# Autodesk Inventor assembly: Full_Auto_Robot_Assembly_V1.1_16.10.25
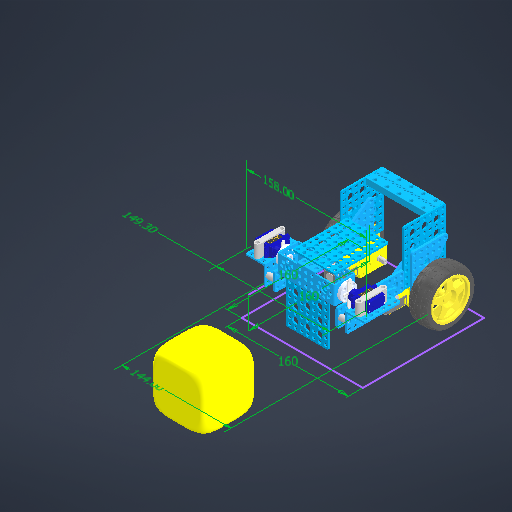
[picture p0: Inventor's stored thumbnail of the model, 512x512]
Saved by Autodesk Inventor 2026.1 (Build 301233020, 233B)
## iProperties
Created: 2025-10-11
Part Number: Full_Auto_Robot_Assembly_V1.1_16.10.25
Document SubType Name: Assembly
Designer: Asus
Author: Asus
## Documents named in this file (13)
- D:\KMITL\Computer_Programming\ComPro_Project\Robot_design_CAD_files\Full_Auto_Robot_Assembly_V1.1_16.10.25.iam
- D:\KMITL\Computer_Programming\ComPro_Project\Material_Parts_CAD_files\Metal_parts\Plate0324-088 V1.0.ipt
- D:\KMITL\Computer_Programming\ComPro_Project\Material_Parts_CAD_files\Metal_parts\Triangle Plate 6x8.ipt
- D:\KMITL\Computer_Programming\ComPro_Project\Material_Parts_CAD_files\Metal_parts\Beam0824-5.ipt
- D:\KMITL\Computer_Programming\ComPro_Project\Material_Parts_CAD_files\Metal_parts\Plate 7x9.ipt
- D:\KMITL\Computer_Programming\ComPro_Project\Material_Parts_CAD_files\Electronic_parts\yellow_dc_motor.ipt
- D:\KMITL\Computer_Programming\ComPro_Project\Material_Parts_CAD_files\Arudino_parts\Wheel D65x25.ipt
- D:\KMITL\Computer_Programming\ComPro_Project\Robot_design_CAD_files\Auto_robot_gate_mechanism_V1_11.10.25.iam
- D:\KMITL\Computer_Programming\ComPro_Project\Material_Parts_CAD_files\Metal_parts\Bracket 3x6.ipt
- D:\KMITL\Computer_Programming\ComPro_Project\Material_Parts_CAD_files\MakeX_parts\Standoff_010.ipt
- D:\KMITL\Computer_Programming\ComPro_Project\Field_materials_CAD_files\Objective_Block_Auto.ipt
- D:\KMITL\Computer_Programming\ComPro_Project\3D_Printing_Parts_CAD_files\Micro_servo_frame_2.ipt
- D:\KMITL\Computer_Programming\ComPro_Project\3D_Printing_Parts_CAD_files\Micro_servo_frame_1.ipt
## Components (25 placed, 12 different names)
1. Plate0324-088 V1.0:1 — Rigid:4, Mate:1, Mate:2, Mate:3, Mate:15, Tangent:1, Mate:18, Rigid:8, Rigid:9
2. Triangle Plate 6x8:1 — Rigid:4, Mate:1, Mate:2, Mate:3, Mate:4, Rigid:1
3. Beam0824-5:1 — Mate:6, Mate:7, Mate:8, Mate:11, Mate:12, Mate:13
4. Plate 7x9:1 — Mate:4, Rigid:1, Mate:5, Rigid:5, Mate:6, Mate:7, Mate:8
5. Triangle Plate 6x8:2 — Mate:5, Rigid:5, Mate:16
6. Plate0324-088 V1.0:2 — Rigid:6, Rigid:11, Rigid:12
7. Triangle Plate 6x8:3 — Rigid:6, Rotational:1, Mate:14
8. Plate 7x9:2 — Rotational:1, Mate:9, Mate:10, Rigid:7, Mate:11, Mate:12, Mate:13, Mate:14
9. Triangle Plate 6x8:4 — Mate:9, Mate:10, Rigid:7, Mate:17
10. yellow_dc_motor:1 — Mate:16, Rotational:2
11. yellow_dc_motor:2 — Mate:17, Rotational:3
12. Wheel D65x25:1 — Rotational:2
13. Wheel D65x25:2 — Rotational:3
14. Auto_robot_gate_mechanism_V1_11.10.25:1 [sub-assembly] — Tangent:1, Mate:18
15. Bracket 3x6:1 — Rigid:10, Rigid:14
16. Standoff_010:1 — Rigid:8, Rigid:10
17. Standoff_010:2 — Rigid:9
18. Standoff_010:3 — Rigid:12
19. Standoff_010:4 — Rigid:11, Rigid:13
20. Bracket 3x6:2 — Rigid:13, Rigid:17
21. Objective_Block_Auto:1 — Mate:19
22. Micro_servo_frame_2:1 — Rigid:14, Rigid:15
23. Micro_servo_frame_2:2 — Rigid:16, Rigid:17
24. Micro_servo_frame_1:1 — Rigid:15
25. Micro_servo_frame_1:2 — Rigid:16
## Relationships (39: Mate 19, WeldJoint 15, RevoluteJoint 3, Flush 1, Tangent 1)
- Rigid:4 [WeldJoint]: Plate0324-088 V1.0:1 ↔ Triangle Plate 6x8:1
- Mate:1: Plate0324-088 V1.0:1 ↔ Triangle Plate 6x8:1
- Mate:2: Plate0324-088 V1.0:1 ↔ Triangle Plate 6x8:1
- Mate:3: Plate0324-088 V1.0:1 ↔ Triangle Plate 6x8:1
- Mate:4: Triangle Plate 6x8:1 ↔ Plate 7x9:1
- Rigid:1 [WeldJoint]: Triangle Plate 6x8:1 ↔ Plate 7x9:1
- Mate:5: Plate 7x9:1 ↔ Triangle Plate 6x8:2
- Rigid:5 [WeldJoint]: Plate 7x9:1 ↔ Triangle Plate 6x8:2
- Mate:6: Beam0824-5:1 ↔ Plate 7x9:1
- Mate:7: Beam0824-5:1 ↔ Plate 7x9:1
- Mate:8: Beam0824-5:1 ↔ Plate 7x9:1
- Rigid:6 [WeldJoint]: Plate0324-088 V1.0:2 ↔ Triangle Plate 6x8:3
- Rotational:1 [RevoluteJoint]: Triangle Plate 6x8:3 ↔ Plate 7x9:2
- Mate:9: Plate 7x9:2 ↔ Triangle Plate 6x8:4
- Mate:10: Plate 7x9:2 ↔ Triangle Plate 6x8:4
- Rigid:7 [WeldJoint]: Plate 7x9:2 ↔ Triangle Plate 6x8:4
- Mate:11: Beam0824-5:1 ↔ Plate 7x9:2
- Mate:12: Beam0824-5:1 ↔ Plate 7x9:2
- Mate:13: Beam0824-5:1 ↔ Plate 7x9:2
- Mate:14: Triangle Plate 6x8:3 ↔ Plate 7x9:2
- Mate:15: Plate0324-088 V1.0:1
- Mate:16: Triangle Plate 6x8:2 ↔ yellow_dc_motor:1
- Mate:17: Triangle Plate 6x8:4 ↔ yellow_dc_motor:2
- Rotational:2 [RevoluteJoint]: yellow_dc_motor:1 ↔ Wheel D65x25:1
- Rotational:3 [RevoluteJoint]: yellow_dc_motor:2 ↔ Wheel D65x25:2
- Flush:1 (-46.5 mm)
- Tangent:1: Plate0324-088 V1.0:1 ↔ Auto_robot_gate_mechanism_V1_11.10.25:1
- Mate:18: Plate0324-088 V1.0:1 ↔ Auto_robot_gate_mechanism_V1_11.10.25:1
- Rigid:8 [WeldJoint]: Plate0324-088 V1.0:1 ↔ Standoff_010:1
- Rigid:9 [WeldJoint]: Plate0324-088 V1.0:1 ↔ Standoff_010:2
- Rigid:10 [WeldJoint]: Bracket 3x6:1 ↔ Standoff_010:1
- Rigid:11 [WeldJoint]: Plate0324-088 V1.0:2 ↔ Standoff_010:4
- Rigid:12 [WeldJoint]: Plate0324-088 V1.0:2 ↔ Standoff_010:3
- Rigid:13 [WeldJoint]: Standoff_010:4 ↔ Bracket 3x6:2
- Mate:19: Objective_Block_Auto:1
- Rigid:14 [WeldJoint]: Bracket 3x6:1 ↔ Micro_servo_frame_2:1
- Rigid:15 [WeldJoint]: Micro_servo_frame_2:1 ↔ Micro_servo_frame_1:1
- Rigid:16 [WeldJoint]: Micro_servo_frame_2:2 ↔ Micro_servo_frame_1:2
- Rigid:17 [WeldJoint]: Bracket 3x6:2 ↔ Micro_servo_frame_2:2
